# Autodesk Inventor assembly: controller
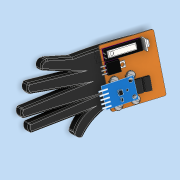
[picture p0: Inventor's stored thumbnail of the model, 180x180]
Saved by Autodesk Inventor 2022 (Build 260153000, 153)
## iProperties
Created: 2021-06-27
Part Number: controller
Document SubType Name: Assembly
Designer: TAMAZZER FAHIM
Author: TAMAZZER FAHIM
## Documents named in this file (6)
- E:\controller2\controller.iam
- E:\controller2\controllerbase.ipt
- E:\controller2\controllerchannel.ipt
- E:\controller2\controllerchannel1.ipt
- E:\controller2\controlleraccelerometer.ipt
- E:\controller2\glove.ipt
## Components (8 placed, 5 different names)
1. controllerbase:1 — Mate:1, Mate:2, Mate:3, Mate:4, Mate:5, Mate:7
2. controllerchannel:1 — Mate:4
3. controllerchannel:2 — Mate:3
4. controllerchannel:3 — Mate:1
5. controllerchannel:4 — Mate:2
6. controllerchannel1:1 — Mate:5, Mate:6
7. controlleraccelerometer:1 — Mate:6
8. glove:1 — Mate:7
## Relationships (7: Mate 7)
- Mate:1: controllerbase:1 ↔ controllerchannel:3
- Mate:2: controllerbase:1 ↔ controllerchannel:4
- Mate:3: controllerbase:1 ↔ controllerchannel:2
- Mate:4: controllerbase:1 ↔ controllerchannel:1
- Mate:5: controllerbase:1 ↔ controllerchannel1:1
- Mate:6: controllerchannel1:1 ↔ controlleraccelerometer:1
- Mate:7: controllerbase:1 ↔ glove:1
